# Autodesk Inventor assembly: 4 in Traction Tire
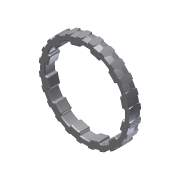
[picture p0: Inventor's stored thumbnail of the model, 180x180]
Saved by Autodesk Inventor 2013 (Build 170138000, 138)
## iProperties
Created: 2013-12-23
Part Number: 4 in Traction Tire
Document SubType Name: Assembly
Designer: Nemo
Author: Nemo
## Documents named in this file (3)
- H:\Nemo\Documents\Robotics\COTS Parts\Wheels\VexPro Traction Wheels\Components\4 in Traction Tire.iam
- H:\Nemo\Documents\Robotics\COTS Parts\Wheels\VexPro Traction Wheels\Components\4 in Traction Tire insert.ipt
- H:\Nemo\Documents\Robotics\COTS Parts\Wheels\VexPro Traction Wheels\Components\4 in Traction Tire Tread.ipt
## Components (2 placed, 2 different names)
1. 4 in Traction Tire insert:1
2. 4 in Traction Tire Tread:1 — Mate:1, Flush:1, Mate:2
## Relationships (3: Mate 2, Flush 1)
- Mate:1: 4 in Traction Tire Tread:1
- Flush:1: 4 in Traction Tire Tread:1
- Mate:2: 4 in Traction Tire Tread:1
